# Autodesk Inventor assembly: 100002
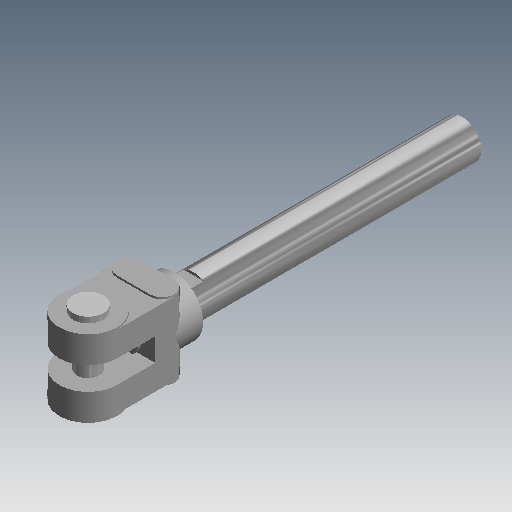
[picture p0: Inventor's stored thumbnail of the model, 512x512]
Saved by Autodesk Inventor 2020.1 (Build 241239000, 239)
## iProperties
Created: 2006-02-02
Part Number: 100002
Document SubType Name: Assembly
Designer: Kevin
Manufacturer: Standard
Standards Organization: Custom
Weld Material: Default
Author: Kevin
## Documents named in this file (4)
- C:\Users\thom_tremblay\Desktop\Inventor ACP Data\Assemblies\PH-000-002.iam
- C:\Users\thom_tremblay\Desktop\Inventor ACP Data\Parts\PH-200-013.ipt
- C:\Users\thom_tremblay\Desktop\Inventor ACP Data\Parts\PH-200-014.ipt
- C:\Users\thom_tremblay\Desktop\Inventor ACP Data\Content Center\en-US\ISO 1234\11-2.5-20.ipt
## Components (3 placed, 3 different names)
1. PH-200-013:1
2. PH-200-014:1 — Mate:1, Tangent:1
3. "ISO 1234" 2.5 x 20:1 — Mate:1, Tangent:1
## Relationships (3: Insert 1, Mate 1, Tangent 1)
- [Insert]: PH-200-013:1 ↔ PH-200-014:1
- Mate:1: PH-200-014:1 ↔ "ISO 1234" 2.5 x 20:1
- Tangent:1: PH-200-014:1 ↔ "ISO 1234" 2.5 x 20:1
